# Autodesk Inventor assembly: 202.002.01_Schieberbetaetigung
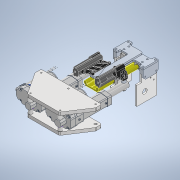
[picture p0: Inventor's stored thumbnail of the model, 180x180]
Saved by Autodesk Inventor 2021 (Build 250183000, 183)
## iProperties
Created: 2021-11-14
Part Number: 202.002.01_Schieberbetaetigung
Document SubType Name: Assembly
Designer: Oliver Ungerer
KODE_ZEICHNUNGSNUMMER: TFVEM_110M
BENENNUNG: Fuehrung Schieber
BEARBEITER_NAME: Ungerer O.
MASSE: 2.190774
PDMREV: 0.0+
PDMRL: Entwicklung
PROI_REVISION: 0
PROI_VERSION: 0+
PROI_RELEASE: Entwicklung
PTC_MODIFIED: True
PROI_CREATED_BY: Kantioler_adm
PROI_CREATED_ON: 07.03.2008 12:11:19
PROI_LOCATION: Root-Ordner/Pro_stds/Start_Files
MATERIALART: -
EINHEIT: ST
HERSTELLER_PREIS: 0.0
PRUEFER_NAME: Uo
PTC_ORGANIZATION_ID: Durst
PTC_WM_REVISION: 0
PTC_WM_ITERATION: 0
PTC_WM_VERSION: 0.0
PTC_WM_LIFECYCLE_STATE: Entwicklung
PTC_WM_LIFECYCLE: 02 Durst
PTC_WM_CREATED_BY: Oliver Ungerer (oungerer: Durst)
PTC_WM_CREATED_ON: 01.08.21
PTC_WM_MODIFIED_BY: Oliver Ungerer (oungerer: Durst)
PTC_WM_MODIFIED_ON: 01.08.21
AEND_INDEX: 0
VERSION: 0
STATUS: 0.0
Author: Oliver Ungerer
## Documents named in this file (21)
- C:\Users\Sebastian Seewald\Documents\Inventor\Konstruktion_Studium\Lernfabrik\106_Vereinzelungseinheit\202.002.01_Schieberbetaetigung.iam
- C:\Users\Sebastian Seewald\Documents\Inventor\Konstruktion_Studium\Lernfabrik\106_Vereinzelungseinheit\0001_IGUS_SCHIENE.ipt
- C:\Users\Sebastian Seewald\Documents\Inventor\Konstruktion_Studium\Lernfabrik\106_Vereinzelungseinheit\1346134.ipt
- C:\Users\Sebastian Seewald\Documents\Inventor\Konstruktion_Studium\Lernfabrik\106_Vereinzelungseinheit\TFVEM_10100.ipt
- C:\Users\Sebastian Seewald\Documents\Inventor\Konstruktion_Studium\Lernfabrik\106_Vereinzelungseinheit\TFVEM_1106.ipt
- C:\Users\Sebastian Seewald\Documents\Inventor\Konstruktion_Studium\Lernfabrik\106_Vereinzelungseinheit\TFVEM_1101.ipt
- C:\Users\Sebastian Seewald\Documents\Inventor\Konstruktion_Studium\Lernfabrik\106_Vereinzelungseinheit\TFVEM_10102.ipt
- C:\Users\Sebastian Seewald\Documents\Inventor\Konstruktion_Studium\Lernfabrik\106_Vereinzelungseinheit\TFVEM_10103.ipt
- C:\Users\Sebastian Seewald\Documents\Inventor\Konstruktion_Studium\Lernfabrik\106_Vereinzelungseinheit\TFVEM_10104.ipt
- C:\Users\Sebastian Seewald\Documents\Inventor\Konstruktion_Studium\Lernfabrik\106_Vereinzelungseinheit\TFVEM_10105.ipt
- C:\Users\Sebastian Seewald\Documents\Inventor\Konstruktion_Studium\Lernfabrik\106_Vereinzelungseinheit\TFVEM_1009.ipt
- C:\Users\Sebastian Seewald\Documents\Inventor\Konstruktion_Studium\Lernfabrik\106_Vereinzelungseinheit\1237347.ipt
- C:\Users\Sebastian Seewald\Documents\Inventor\Konstruktion_Studium\Lernfabrik\106_Vereinzelungseinheit\1126405.ipt
- C:\Users\Sebastian Seewald\Documents\Inventor\Konstruktion_Studium\Lernfabrik\106_Vereinzelungseinheit\1126767.ipt
- C:\Users\Sebastian Seewald\Documents\Inventor\Konstruktion_Studium\Lernfabrik\106_Vereinzelungseinheit\202.003.01_Kraftlimitierung.iam
- C:\Users\Sebastian Seewald\Documents\Inventor\Konstruktion_Studium\Lernfabrik\106_Vereinzelungseinheit\202.004.01_Kraftlimitierung.iam
- C:\Users\Sebastian Seewald\Documents\Inventor\Konstruktion_Studium\Lernfabrik\106_Vereinzelungseinheit\502.001.01_Linearaktor.iam
- C:\Users\Sebastian Seewald\Documents\Inventor\Konstruktion_Studium\Lernfabrik\106_Vereinzelungseinheit\202.006.01_Anbindung_Aktor.ipt
- C:\Users\Sebastian Seewald\Documents\Inventor\Konstruktion_Studium\Lernfabrik\106_Vereinzelungseinheit\102.004.01_Zapfen_Aktor.ipt
- C:\Users\Sebastian Seewald\Documents\Inventor\Konstruktion_Studium\Lernfabrik\106_Vereinzelungseinheit\102.005.01_Zapfen_Aktor_Auflage.ipt
- C:\Users\Sebastian Seewald\Documents\Inventor\Konstruktion_Studium\Lernfabrik\106_Vereinzelungseinheit\102.006.01_Anbindung_Aktor.ipt
## Components (31 placed, 19 different names)
1. 506.004.01_IGUS_Schiene — Fluchtend:1, Passend:15, Winkel:1, Passend:20, Winkel:2, Fluchtend:2, Passend:21, Winkel:3, Passend:23, Winkel:4
2. 106.015.01_Schienenfuehrung — Fluchtend:1, Passend:15, Winkel:1, Passend:16, Passend:17, Passend:18, Passend:19
3. 106.015.01_Schienenfuehrung:1 — Passend:22, Passend:23, Winkel:4, Passend:24, Passend:25, Passend:26
4. 106.015.01_Schienenfuehrung:2 — Fluchtend:2, Passend:21, Winkel:3, Passend:22, Passend:30, Passend:32
5. 106.015.01_Schienenfuehrung:3 — Passend:19, Passend:20, Winkel:2, Passend:31
6. 106.016.01_Distanzstueck — Passend:16, Passend:17, Passend:18, Passend:27, Passend:29
7. 106.017.01_Zwischenstueck_Schieber_oben — Passend:27, Passend:28, Passend:29, Passend:36, Passend:37, Passend:38, Passend:78, Passend:79, Passend:80
8. 106.018.01_Zwischenstueck_Schieber_unten — Passend:30, Passend:31, Passend:32, Passend:33, Passend:34, Passend:35, Passend:74, Passend:75, Passend:76
9. 106.016.01_Distanzstueck:1 — Passend:24, Passend:25, Passend:26, Passend:28
10. 106.017.01_Aufnahme_Schwert — Passend:36, Passend:37, Passend:38, Passend:42, Passend:43, Passend:44
11. 106.018.01_Schwert_oben — Passend:42, Passend:43, Passend:44
12. 106.017.01_Aufnahme_Schwert:1 — Passend:33, Passend:34, Passend:35, Passend:39, Passend:40, Passend:41
13. 106.019.01_Schwert_unten — Passend:39, Passend:40, Passend:41
14. 202.003.01_Kraftlimitierung:1 [sub-assembly] — Passend:74, Passend:75, Passend:76, Passend:77
15. 202.004.01_Kraftlimitierung:1 [sub-assembly] — Passend:78, Passend:79, Passend:80, Passend:81
16. 106.020.01_Distanzbolzen_groß — Passend:61, Passend:63, Passend:64, Passend:65, Passend:81, Passend:87
17. 106.021.01_Distanzbolzen_klein — Passend:55, Passend:56, Passend:57, Passend:77, Passend:83
18. 106.022.01_Unterlegscheibe — Passend:55, Passend:56, Passend:58
19. 106.022.01_Unterlegscheibe:1 — Passend:63, Passend:64, Passend:66
20. DIN_9012_M4x8 — Passend:65, Passend:66
21. DIN_9012_M4x8:1 — Passend:57, Passend:58
22. DIN_9012_M4x12
23. DIN_9012_M4x12:1 — Passend:61
24. 106.023.01_Zapfen_Aktor:1 — Passend:7, Passend:8, Passend:71, Passend:86
25. 106.023.01_Zapfen_Aktor:2 — Passend:5, Passend:6, Passend:72, Passend:73, Passend:82, Passend:84
26. 106.024.01_Zapfen_Aktor_Auflage:1 — Passend:7, Passend:8
27. 106.024.01_Zapfen_Aktor_Auflage:2 — Passend:5, Passend:6
28. 106.025.01_Anbindung_Aktor:1 — Passend:71, Passend:72, Passend:73
29. 106.025.01_Anbindung_Aktor:2
30. 506.005.01_Linearaktor:1 [sub-assembly] — Passend:82, Passend:83, Passend:84, Passend:85, Fluchtend:3, Winkel:5
31. 506.005.01_Linearaktor:2 [sub-assembly] — Passend:86, Passend:87, Fluchtend:3
## Relationships (71: Mate 63, Angle 5, Flush 3)
- Passend:5 [Mate]: 106.023.01_Zapfen_Aktor:2 ↔ 106.024.01_Zapfen_Aktor_Auflage:2
- Passend:6 [Mate]: 106.023.01_Zapfen_Aktor:2 ↔ 106.024.01_Zapfen_Aktor_Auflage:2
- Passend:7 [Mate]: 106.023.01_Zapfen_Aktor:1 ↔ 106.024.01_Zapfen_Aktor_Auflage:1
- Passend:8 [Mate]: 106.023.01_Zapfen_Aktor:1 ↔ 106.024.01_Zapfen_Aktor_Auflage:1
- [Mate]: 106.024.01_Zapfen_Aktor_Auflage:2 ↔ 106.025.01_Anbindung_Aktor:2
- [Mate]: 106.024.01_Zapfen_Aktor_Auflage:1 ↔ 106.025.01_Anbindung_Aktor:2
- [Mate]: 106.024.01_Zapfen_Aktor_Auflage:2 ↔ 106.025.01_Anbindung_Aktor:2
- Fluchtend:1 [Flush] (0.5 mm): 506.004.01_IGUS_Schiene ↔ 106.015.01_Schienenfuehrung
- Passend:15 [Mate]: 506.004.01_IGUS_Schiene ↔ 106.015.01_Schienenfuehrung
- Winkel:1 [Angle] (0 deg): 506.004.01_IGUS_Schiene ↔ 106.015.01_Schienenfuehrung
- Passend:16 [Mate]: 106.015.01_Schienenfuehrung ↔ 106.016.01_Distanzstueck
- Passend:17 [Mate]: 106.015.01_Schienenfuehrung ↔ 106.016.01_Distanzstueck
- Passend:18 [Mate]: 106.015.01_Schienenfuehrung ↔ 106.016.01_Distanzstueck
- Passend:19 [Mate] (51 mm): 106.015.01_Schienenfuehrung ↔ 106.015.01_Schienenfuehrung:3
- Passend:20 [Mate]: 506.004.01_IGUS_Schiene ↔ 106.015.01_Schienenfuehrung:3
- Winkel:2 [Angle] (0 deg): 506.004.01_IGUS_Schiene ↔ 106.015.01_Schienenfuehrung:3
- Fluchtend:2 [Flush] (0.5 mm): 506.004.01_IGUS_Schiene ↔ 106.015.01_Schienenfuehrung:2
- Passend:21 [Mate]: 506.004.01_IGUS_Schiene ↔ 106.015.01_Schienenfuehrung:2
- Winkel:3 [Angle] (0 deg): 506.004.01_IGUS_Schiene ↔ 106.015.01_Schienenfuehrung:2
- Passend:22 [Mate] (51 mm): 106.015.01_Schienenfuehrung:1 ↔ 106.015.01_Schienenfuehrung:2
- Passend:23 [Mate]: 506.004.01_IGUS_Schiene ↔ 106.015.01_Schienenfuehrung:1
- Winkel:4 [Angle] (0 deg): 506.004.01_IGUS_Schiene ↔ 106.015.01_Schienenfuehrung:1
- Passend:24 [Mate]: 106.015.01_Schienenfuehrung:1 ↔ 106.016.01_Distanzstueck:1
- Passend:25 [Mate]: 106.015.01_Schienenfuehrung:1 ↔ 106.016.01_Distanzstueck:1
- Passend:26 [Mate]: 106.015.01_Schienenfuehrung:1 ↔ 106.016.01_Distanzstueck:1
- Passend:27 [Mate]: 106.016.01_Distanzstueck ↔ 106.017.01_Zwischenstueck_Schieber_oben
- Passend:28 [Mate]: 106.017.01_Zwischenstueck_Schieber_oben ↔ 106.016.01_Distanzstueck:1
- Passend:29 [Mate]: 106.016.01_Distanzstueck ↔ 106.017.01_Zwischenstueck_Schieber_oben
- Passend:30 [Mate]: 106.015.01_Schienenfuehrung:2 ↔ 106.018.01_Zwischenstueck_Schieber_unten
- Passend:31 [Mate]: 106.015.01_Schienenfuehrung:3 ↔ 106.018.01_Zwischenstueck_Schieber_unten
- Passend:32 [Mate]: 106.015.01_Schienenfuehrung:2 ↔ 106.018.01_Zwischenstueck_Schieber_unten
- Passend:33 [Mate]: 106.018.01_Zwischenstueck_Schieber_unten ↔ 106.017.01_Aufnahme_Schwert:1
- Passend:34 [Mate]: 106.018.01_Zwischenstueck_Schieber_unten ↔ 106.017.01_Aufnahme_Schwert:1
- Passend:35 [Mate]: 106.018.01_Zwischenstueck_Schieber_unten ↔ 106.017.01_Aufnahme_Schwert:1
- Passend:36 [Mate]: 106.017.01_Zwischenstueck_Schieber_oben ↔ 106.017.01_Aufnahme_Schwert
- Passend:37 [Mate]: 106.017.01_Zwischenstueck_Schieber_oben ↔ 106.017.01_Aufnahme_Schwert
- Passend:38 [Mate]: 106.017.01_Zwischenstueck_Schieber_oben ↔ 106.017.01_Aufnahme_Schwert
- Passend:39 [Mate]: 106.017.01_Aufnahme_Schwert:1 ↔ 106.019.01_Schwert_unten
- Passend:40 [Mate]: 106.017.01_Aufnahme_Schwert:1 ↔ 106.019.01_Schwert_unten
- Passend:41 [Mate]: 106.017.01_Aufnahme_Schwert:1 ↔ 106.019.01_Schwert_unten
- Passend:42 [Mate]: 106.017.01_Aufnahme_Schwert ↔ 106.018.01_Schwert_oben
- Passend:43 [Mate]: 106.017.01_Aufnahme_Schwert ↔ 106.018.01_Schwert_oben
- Passend:44 [Mate]: 106.017.01_Aufnahme_Schwert ↔ 106.018.01_Schwert_oben
- Passend:55 [Mate]: 106.021.01_Distanzbolzen_klein ↔ 106.022.01_Unterlegscheibe
- Passend:56 [Mate]: 106.021.01_Distanzbolzen_klein ↔ 106.022.01_Unterlegscheibe
- Passend:57 [Mate]: 106.021.01_Distanzbolzen_klein ↔ DIN_9012_M4x8:1
- Passend:58 [Mate]: 106.022.01_Unterlegscheibe ↔ DIN_9012_M4x8:1
- Passend:61 [Mate]: 106.020.01_Distanzbolzen_groß ↔ DIN_9012_M4x12:1
- Passend:63 [Mate]: 106.020.01_Distanzbolzen_groß ↔ 106.022.01_Unterlegscheibe:1
- Passend:64 [Mate]: 106.020.01_Distanzbolzen_groß ↔ 106.022.01_Unterlegscheibe:1
- Passend:65 [Mate]: 106.020.01_Distanzbolzen_groß ↔ DIN_9012_M4x8
- Passend:66 [Mate]: 106.022.01_Unterlegscheibe:1 ↔ DIN_9012_M4x8
- Passend:71 [Mate]: 106.023.01_Zapfen_Aktor:1 ↔ 106.025.01_Anbindung_Aktor:1
- Passend:72 [Mate]: 106.023.01_Zapfen_Aktor:2 ↔ 106.025.01_Anbindung_Aktor:1
- Passend:73 [Mate]: 106.023.01_Zapfen_Aktor:2 ↔ 106.025.01_Anbindung_Aktor:1
- Passend:74 [Mate]: 106.018.01_Zwischenstueck_Schieber_unten ↔ 202.003.01_Kraftlimitierung:1
- Passend:75 [Mate]: 106.018.01_Zwischenstueck_Schieber_unten ↔ 202.003.01_Kraftlimitierung:1
- Passend:76 [Mate]: 106.018.01_Zwischenstueck_Schieber_unten ↔ 202.003.01_Kraftlimitierung:1
- Passend:77 [Mate]: 202.003.01_Kraftlimitierung:1 ↔ 106.021.01_Distanzbolzen_klein
- Passend:78 [Mate]: 106.017.01_Zwischenstueck_Schieber_oben ↔ 202.004.01_Kraftlimitierung:1
- Passend:79 [Mate]: 106.017.01_Zwischenstueck_Schieber_oben ↔ 202.004.01_Kraftlimitierung:1
- Passend:80 [Mate]: 106.017.01_Zwischenstueck_Schieber_oben ↔ 202.004.01_Kraftlimitierung:1
- Passend:81 [Mate]: 202.004.01_Kraftlimitierung:1 ↔ 106.020.01_Distanzbolzen_groß
- Passend:82 [Mate]: 106.023.01_Zapfen_Aktor:2 ↔ 506.005.01_Linearaktor:1
- Passend:83 [Mate]: 106.021.01_Distanzbolzen_klein ↔ 506.005.01_Linearaktor:1
- Passend:84 [Mate] (1 mm): 106.023.01_Zapfen_Aktor:2 ↔ 506.005.01_Linearaktor:1
- Passend:85 [Mate] (-3 mm): 506.005.01_Linearaktor:1
- Passend:86 [Mate]: 106.023.01_Zapfen_Aktor:1 ↔ 506.005.01_Linearaktor:2
- Passend:87 [Mate]: 106.020.01_Distanzbolzen_groß ↔ 506.005.01_Linearaktor:2
- Fluchtend:3 [Flush]: 506.005.01_Linearaktor:1 ↔ 506.005.01_Linearaktor:2
- Winkel:5 [Angle] (180 deg): 506.005.01_Linearaktor:1
## Named parameters: d11_d6 = 0 mm, d12_d7 = 0 mm
